# Autodesk Inventor assembly: Robot
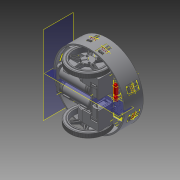
[picture p0: Inventor's stored thumbnail of the model, 180x180]
Saved by Autodesk Inventor 2014 (Build 180170000, 170)
## iProperties
Created: 2013-06-25
Part Number: Robot
Document SubType Name: Assembly
Designer: Felix
Author: Felix
## Documents named in this file (8)
- C:\Users\Felix\Desktop\Beep\Hardware\3D-CAD\Robot.iam
- C:\Users\Felix\Desktop\Beep\Hardware\3D-CAD\parts\Pololu_gear_motor_1_180\gear_motor.iam
- C:\Users\Felix\Desktop\Beep\Hardware\3D-CAD\parts\Pololu_Wheel_6mm\Wheel.iam
- C:\Users\Felix\Desktop\Beep\Hardware\3D-CAD\parts\battery_holder\holder_with_batteries_18500.iam
- C:\Users\Felix\Desktop\Beep\Hardware\3D-CAD\parts\battery_holder\holder_with_batteries_18650.iam
- C:\Users\Felix\Desktop\Beep\Hardware\3D-CAD\case\base.ipt
- C:\Users\Felix\Desktop\Beep\Hardware\3D-CAD\parts\electronic\pcb_assembly.iam
- C:\Users\Felix\Desktop\Beep\Hardware\3D-CAD\parts\electronic\BEEP\beep_rgb_ir_assembled.iam
## Components (10 placed, 7 different names)
1. gear_motor:1 [sub-assembly] — Passend:1, Passend:5, Passend:6, Passend:7, Fluchtend:3, Passend:13, Passend:14, Passend:16, Passend:18, Passend:19, Passend:24
2. gear_motor:2 [sub-assembly] — Passend:1, Passend:2, Passend:3, Passend:4, Fluchtend:3, Fluchtend:4, Fluchtend:5, Passend:12, Passend:15
3. Wheel:1 [sub-assembly] — Passend:5, Passend:6, Passend:7, Passend:24
4. Wheel:2 [sub-assembly] — Passend:2, Passend:3, Passend:4
5. holder_with_batteries_18500:1 [sub-assembly] — Fluchtend:4, Passend:13, Passend:14, Passend:15, Fluchtend:6
6. holder_with_batteries_18650:1 [sub-assembly] — Fluchtend:5, Passend:12, Passend:16
7. base:1 — Fluchtend:6, Passend:26, Passend:27, Passend:28, Fluchtend:7, Fluchtend:8, Fluchtend:9, Fluchtend:10, Fluchtend:11
8. pcb_assembly:1 [sub-assembly] — Passend:26, Passend:27, Passend:28, Fluchtend:7, Fluchtend:8, Fluchtend:9, Fluchtend:10, Fluchtend:11
9. beep_rgb_ir_assembled:1 [sub-assembly]
10. beep_rgb_ir_assembled:2 [sub-assembly]
## Relationships (27: Mate 18, Flush 9)
- Passend:1 [Mate]: gear_motor:1 ↔ gear_motor:2
- Passend:2 [Mate]: gear_motor:2 ↔ Wheel:2
- Passend:3 [Mate]: gear_motor:2 ↔ Wheel:2
- Passend:4 [Mate]: gear_motor:2 ↔ Wheel:2
- Passend:5 [Mate]: gear_motor:1 ↔ Wheel:1
- Passend:6 [Mate]: gear_motor:1 ↔ Wheel:1
- Passend:7 [Mate]: gear_motor:1 ↔ Wheel:1
- Fluchtend:3 [Flush]: gear_motor:1 ↔ gear_motor:2
- Fluchtend:4 [Flush]: gear_motor:2 ↔ holder_with_batteries_18500:1
- Fluchtend:5 [Flush]: gear_motor:2 ↔ holder_with_batteries_18650:1
- Passend:12 [Mate]: gear_motor:2 ↔ holder_with_batteries_18650:1
- Passend:13 [Mate]: gear_motor:1 ↔ holder_with_batteries_18500:1
- Passend:14 [Mate]: gear_motor:1 ↔ holder_with_batteries_18500:1
- Passend:15 [Mate]: gear_motor:2 ↔ holder_with_batteries_18500:1
- Passend:16 [Mate]: gear_motor:1 ↔ holder_with_batteries_18650:1
- Passend:18 [Mate]: gear_motor:1
- Passend:19 [Mate]: gear_motor:1
- Passend:24 [Mate]: gear_motor:1 ↔ Wheel:1
- Fluchtend:6 [Flush]: holder_with_batteries_18500:1 ↔ base:1
- Passend:26 [Mate]: base:1 ↔ pcb_assembly:1
- Passend:27 [Mate]: base:1 ↔ pcb_assembly:1
- Passend:28 [Mate]: base:1 ↔ pcb_assembly:1
- Fluchtend:7 [Flush]: base:1 ↔ pcb_assembly:1
- Fluchtend:8 [Flush]: base:1 ↔ pcb_assembly:1
- Fluchtend:9 [Flush]: base:1 ↔ pcb_assembly:1
- Fluchtend:10 [Flush]: base:1 ↔ pcb_assembly:1
- Fluchtend:11 [Flush]: base:1 ↔ pcb_assembly:1
